# Autodesk Inventor assembly: MX-106T_bottom
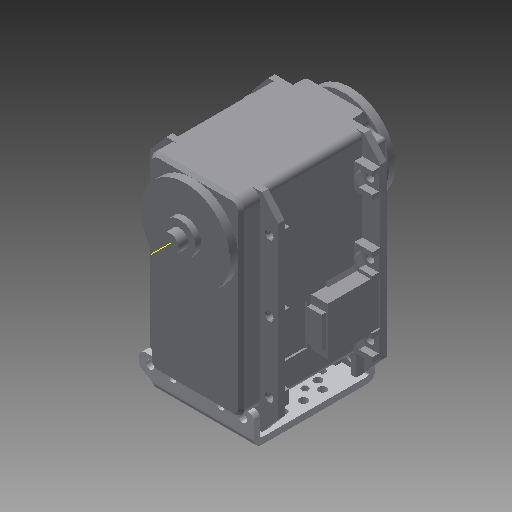
[picture p0: Inventor's stored thumbnail of the model, 512x512]
Saved by Autodesk Inventor 2018 (Build 220112000, 112)
## iProperties
Created: 2017-02-17
Part Number: MX-106T_bottom
Document SubType Name: Assembly
Designer: steve
Mass: 166.177 g
Surface Area: 225.605 cm^2
Volume: 90.7516 cm^3
Density: 1.83112 g/cm^3
Author: steve
## Documents named in this file (6)
- C:\Users\medrimonia\Dropbox\SigmaBan\SigmaBanV2.1\MX-106T_bottom.iam
- C:\Users\medrimonia\Dropbox\SigmaBan\SigmaBanV2.1\MX-106T.ipt
- C:\Users\medrimonia\Dropbox\SigmaBan\SigmaBanV2.1\FR05-S101.ipt
- C:\Users\medrimonia\Dropbox\SigmaBan\SigmaBanV2.1\RX64-CAP.ipt
- C:\Users\medrimonia\Dropbox\SigmaBan\SigmaBanV2.1\dynamixel\horn\HN05-i101.ipt
- C:\Users\medrimonia\Dropbox\SigmaBan\SigmaBanV2.1\MF128ZZ.ipt
## Components (5 placed, 5 different names)
1. MX-106T:1 — Mate:1, Mate:2, Mate:3, Mate:8, Mate:9
2. FR05-S101:1 — Mate:1, Mate:2, Mate:3
3. RX64-CAP:1
4. HN05-i101:1
5. MF128ZZ:1 — Mate:8, Mate:9
## Relationships (9: Mate 9)
- Mate:1: MX-106T:1 ↔ FR05-S101:1
- Mate:2: MX-106T:1 ↔ FR05-S101:1
- Mate:3: MX-106T:1 ↔ FR05-S101:1
- [Mate]: HN05-i101:1 ↔ MF128ZZ:1
- [Mate]: RX64-CAP:1 ↔ MF128ZZ:1
- [Mate]: RX64-CAP:1 ↔ MF128ZZ:1
- [Mate]: HN05-i101:1 ↔ MF128ZZ:1
- Mate:8: MX-106T:1 ↔ MF128ZZ:1
- Mate:9: MX-106T:1 ↔ MF128ZZ:1
## Named parameters: d28_d26 = 0 mm, d29_d27 = 0 mm
